# Autodesk Inventor assembly: Wankel_Ricea f. Florentina alexandra-T7
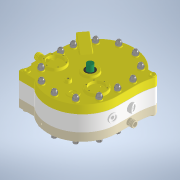
[picture p0: Inventor's stored thumbnail of the model, 180x180]
Saved by Autodesk Inventor 2022 (Build 260153000, 153)
## iProperties
Created: 2022-02-18
Part Number: Wankel_Ricea f. Florentina alexandra-T7
Document SubType Name: Assembly
Designer: mtrot
Unghi: 0,00 deg
Author: mtrot
## Documents named in this file (9)
- C:\1.GAC\Tema7\Wankel_Ricea f. Florentina alexandra-T7.iam
- C:\1.GAC\Tema7\CapacSpate.ipt
- C:\1.GAC\Tema7\StatorWankel.ipt
- C:\1.GAC\Tema7\Arbore.ipt
- C:\1.GAC\Tema7\SansRotor_Ricea f. Florentina alexandra-T7.iam
- C:\1.GAC\Tema7\SansCapacFata_Ricea f. Florentina alexandra-T7.iam
- C:\1.GAC\Tema7\Ans Suruburi Fixare.iam
- C:\1.GAC\Tema7\Ans Piulite Fixare.iam
- C:\Users\Alexandra\Documents\Inventor\Content Center Files\R2022\en-US\ISO 6194 1  T 1\ISO 6194_1 - Type1 22 x 35 x 7.ipt
## Components (9 placed, 8 different names)
1. CapacSpate:1 — Mate:1, Mate:2, Angle:1, Mate:3, Mate:4, Mate:5, Mate:10
2. StatorWankel:1 — Mate:1, Mate:2, Angle:1, Unghi Animatie, Mate:7, Mate:9
3. Arbore:1 — Mate:3, Mate:4, Unghi Animatie, Mate:6, Angle:3, Rotation:1, Mate:8, Mate:11, Mate:13
4. SansRotor_Ricea f. Florentina alexandra-T7:1 [sub-assembly] — Mate:5, Mate:6, Angle:3, Rotation:1
5. SansCapacFata_Ricea f. Florentina alexandra-T7:1 [sub-assembly] — Mate:7, Mate:8, Mate:9, Mate:12
6. Ans Suruburi Fixare:1 [sub-assembly]
7. Ans Piulite Fixare:1 [sub-assembly]
8. ISO 6194/1 Type 1 Type1 22 x 35 x 7:1 — Mate:10, Mate:11
9. ISO 6194/1 Type 1 Type1 22 x 35 x 7:2 — Mate:12, Mate:13
## Relationships (19: Mate 13, Angle 3, Insert 2, RelateRotation 1)
- Mate:1: CapacSpate:1 ↔ StatorWankel:1
- Mate:2: CapacSpate:1 ↔ StatorWankel:1
- Angle:1 (0 deg): CapacSpate:1 ↔ StatorWankel:1
- Mate:3 (1 mm): CapacSpate:1 ↔ Arbore:1
- Mate:4: CapacSpate:1 ↔ Arbore:1
- Unghi Animatie [Angle] (0 deg): StatorWankel:1 ↔ Arbore:1
- Mate:5: CapacSpate:1 ↔ SansRotor_Ricea f. Florentina alexandra-T7:1
- Mate:6: Arbore:1 ↔ SansRotor_Ricea f. Florentina alexandra-T7:1
- Angle:3 (0 deg): Arbore:1 ↔ SansRotor_Ricea f. Florentina alexandra-T7:1
- Rotation:1 [RelateRotation] (3 ul): Arbore:1 ↔ SansRotor_Ricea f. Florentina alexandra-T7:1
- Mate:7: StatorWankel:1 ↔ SansCapacFata_Ricea f. Florentina alexandra-T7:1
- Mate:8: Arbore:1 ↔ SansCapacFata_Ricea f. Florentina alexandra-T7:1
- Mate:9: StatorWankel:1 ↔ SansCapacFata_Ricea f. Florentina alexandra-T7:1
- [Insert]: SansCapacFata_Ricea f. Florentina alexandra-T7:1 ↔ Ans Suruburi Fixare:1
- [Insert]: CapacSpate:1 ↔ Ans Piulite Fixare:1
- Mate:10: CapacSpate:1 ↔ ISO 6194/1 Type 1 Type1 22 x 35 x 7:1
- Mate:11: Arbore:1 ↔ ISO 6194/1 Type 1 Type1 22 x 35 x 7:1
- Mate:12: SansCapacFata_Ricea f. Florentina alexandra-T7:1 ↔ ISO 6194/1 Type 1 Type1 22 x 35 x 7:2
- Mate:13: Arbore:1 ↔ ISO 6194/1 Type 1 Type1 22 x 35 x 7:2
